# Autodesk Inventor assembly: #Turret
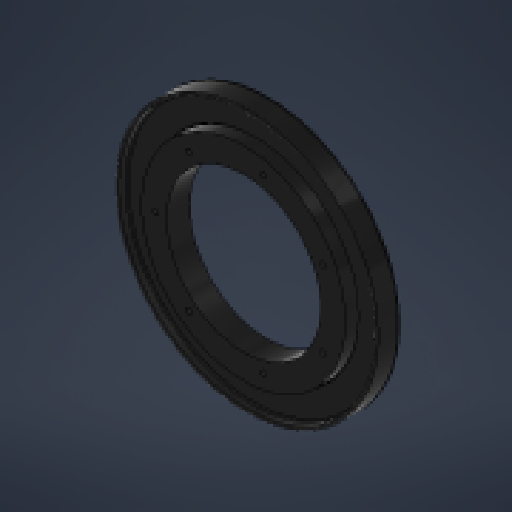
[picture p0: Inventor's stored thumbnail of the model, 512x512]
Saved by Autodesk Inventor 2026.1 (Build 301233020, 233B)
## iProperties
Created: 2026-02-01
Part Number: #Turret
Document SubType Name: Assembly
Designer: Owen L
Mass: 661.765 g
Surface Area: 1768.58 cm^2
Volume: 441.737 cm^3
Density: 1.4981 g/cm^3
Author: Owen L
## Documents named in this file (4)
- C:\Users\Owen\Documents\GitHub\2026-Robot-Mechanical\Shooter\Turret\#Turret.iam
- C:\Users\Owen\Documents\GitHub\2026-Robot-Mechanical\Shooter\Turret\3DPRINT,TURRET,BEARING,INNER.ipt
- C:\Users\Owen\Documents\GitHub\2026-Robot-Mechanical\Shooter\Turret\3DPRINT,TURRET,BEARING,OUTER.ipt
- C:\Users\Owen\Documents\GitHub\2026-Robot-Mechanical\Shooter\Turret\3DPRINT,TURRET,SPACER.ipt
## Components (3 placed, 3 different names)
1. 3DPRINT,TURRET,BEARING,INNER:1 — Flush:1, Mate:1
2. 3DPRINT,TURRET,BEARING,OUTER:1 — Flush:1, Mate:1, Mate:3, Mate:4, Mate:5
3. 3DPRINT,TURRET,SPACER:1 — Mate:3, Mate:4, Mate:5
## Relationships (5: Mate 4, Flush 1)
- Flush:1: 3DPRINT,TURRET,BEARING,INNER:1 ↔ 3DPRINT,TURRET,BEARING,OUTER:1
- Mate:1: 3DPRINT,TURRET,BEARING,INNER:1 ↔ 3DPRINT,TURRET,BEARING,OUTER:1
- Mate:3: 3DPRINT,TURRET,BEARING,OUTER:1 ↔ 3DPRINT,TURRET,SPACER:1
- Mate:4: 3DPRINT,TURRET,BEARING,OUTER:1 ↔ 3DPRINT,TURRET,SPACER:1
- Mate:5: 3DPRINT,TURRET,BEARING,OUTER:1 ↔ 3DPRINT,TURRET,SPACER:1
